# Autodesk Inventor assembly: wheel_assembly
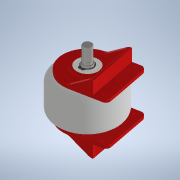
[picture p0: Inventor's stored thumbnail of the model, 180x180]
Saved by Autodesk Inventor 2021.3 (Build 253353000, 353)
## iProperties
Created: 2021-10-12
Part Number: wheel_assembly
Document SubType Name: Assembly
Designer: nxf77172
Author: nxf77172
## Documents named in this file (6)
- C:\Users\nxf77172\Desktop\mechanical_cleaned\custom_parts\drivetrain\wheel_assembly.iam
- C:\Users\nxf77172\Desktop\mechanical_cleaned\custom_parts\drivetrain\wheel_stand_in.ipt
- C:\Users\nxf77172\Desktop\mechanical_cleaned\custom_parts\drivetrain\wheel_axle_mount_plate.ipt
- C:\Users\nxf77172\Desktop\mechanical_cleaned\custom_parts\drivetrain\6003ZZ\AIS2021\SKF_6003-2Z.iam
- C:\Users\nxf77172\Desktop\mechanical_cleaned\custom_parts\drivetrain\wheel_axle\AIS2020\KZBN17-113-P14-LA25-TC4-TB4-KB21-HB50-ZA3-HA18-AA120.iam
- C:\Users\nxf77172\Desktop\mechanical_cleaned\custom_parts\drivetrain\wheel spacer.ipt
## Components (8 placed, 5 different names)
1. wheel_stand_in:1 — Angle:1, Mate:14, Mate:17, Mate:20, Mate:22, Insert:1
2. wheel_axle_mount_plate:1 — Mate:9, Flush:2, Angle:2, Mate:19
3. wheel_axle_mount_plate:2 — Angle:1, Mate:8, Flush:1, Angle:2, Mate:14
4. SKF_6003-2Z:1 [sub-assembly] — Mate:8, Flush:1, Mate:15, Mate:18
5. SKF_6003-2Z:2 [sub-assembly] — Mate:9, Flush:2, Mate:16
6. KZBN17-113-P14-LA25-TC4-TB4-KB21-HB50-ZA3-HA18-AA120:1 [sub-assembly] — Mate:15, Mate:16, Mate:17, Mate:18, Mate:19, Mate:21
7. wheel spacer:1 — Mate:20, Mate:21
8. wheel spacer:2 — Mate:22, Insert:1
## Relationships (16: Mate 11, Angle 2, Flush 2, Insert 1)
- Angle:1 (0 deg): wheel_stand_in:1 ↔ wheel_axle_mount_plate:2
- Mate:8: wheel_axle_mount_plate:2 ↔ SKF_6003-2Z:1
- Flush:1: wheel_axle_mount_plate:2 ↔ SKF_6003-2Z:1
- Mate:9: wheel_axle_mount_plate:1 ↔ SKF_6003-2Z:2
- Flush:2: wheel_axle_mount_plate:1 ↔ SKF_6003-2Z:2
- Angle:2 (0 deg): wheel_axle_mount_plate:1 ↔ wheel_axle_mount_plate:2
- Mate:14 (3 mm): wheel_stand_in:1 ↔ wheel_axle_mount_plate:2
- Mate:15: SKF_6003-2Z:1 ↔ KZBN17-113-P14-LA25-TC4-TB4-KB21-HB50-ZA3-HA18-AA120:1
- Mate:16: SKF_6003-2Z:2 ↔ KZBN17-113-P14-LA25-TC4-TB4-KB21-HB50-ZA3-HA18-AA120:1
- Mate:17: wheel_stand_in:1 ↔ KZBN17-113-P14-LA25-TC4-TB4-KB21-HB50-ZA3-HA18-AA120:1
- Mate:18: SKF_6003-2Z:1 ↔ KZBN17-113-P14-LA25-TC4-TB4-KB21-HB50-ZA3-HA18-AA120:1
- Mate:19: wheel_axle_mount_plate:1 ↔ KZBN17-113-P14-LA25-TC4-TB4-KB21-HB50-ZA3-HA18-AA120:1
- Mate:20: wheel_stand_in:1 ↔ wheel spacer:1
- Mate:21: KZBN17-113-P14-LA25-TC4-TB4-KB21-HB50-ZA3-HA18-AA120:1 ↔ wheel spacer:1
- Mate:22: wheel_stand_in:1 ↔ wheel spacer:2
- Insert:1: wheel_stand_in:1 ↔ wheel spacer:2
